# Autodesk Inventor assembly: RS-380
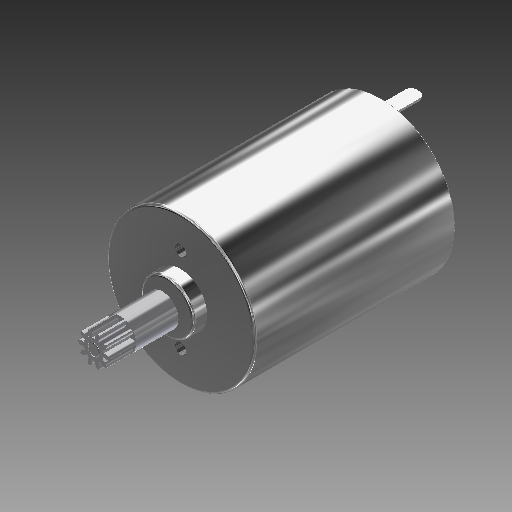
[picture p0: Inventor's stored thumbnail of the model, 512x512]
Saved by Autodesk Inventor 2020 (Build 240168000, 168)
## iProperties
Part Number: RS-380
Material: 一般
Document SubType Name: Assembly
Designer: 雪村
Mass: 85 g
Surface Area: 53.616 cm^2
Volume: 23.992 cm^3
Density: 3.54285 g/cm^3
Description: アセンブリ
Author: 雪村
## Documents named in this file (3)
- C:\Users\white\Documents\SRDC\SRDC\Inventor_2017\2018年機体\パーツ\RS-380.iam
- C:\Users\white\Documents\SRDC\SRDC\Inventor_2017\2018年機体\パーツ\RS-380.ipt
- C:\Users\white\Documents\SRDC\SRDC\Inventor_2017\2018年機体\パーツ\ピニオン10.ipt
## Components (2 placed, 2 different names)
1. RS-380:1 — 挿入:1
2. ピニオン10:1 — 挿入:1
## Relationships (1: Insert 1)
- 挿入:1 [Insert]: RS-380:1 ↔ ピニオン10:1
